# Autodesk Inventor assembly: 05-0010
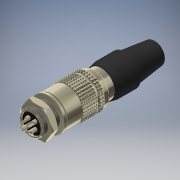
[picture p0: Inventor's stored thumbnail of the model, 180x180]
Saved by Autodesk Inventor 2018 (Build 220112000, 112)
## iProperties
Created: 2019-09-26
Part Number: 05-0010
Document SubType Name: Assembly
Designer: Bradley
Author: Bradley
## Documents named in this file (4)
- C:\Users\Bradley\Documents\GitHub\Resources\SupplierDocuments\05 - Connectors THT\05-0010\05-0010.iam
- C:\Users\Bradley\Documents\GitHub\Resources\SupplierDocuments\05 - Connectors THT\05-0010\05-0010.ipt
- C:\Users\Bradley\Documents\GitHub\Resources\SupplierDocuments\05 - Connectors THT\05-0010P\05-0010P.ipt
- C:\Users\Bradley\Documents\GitHub\Resources\SupplierDocuments\05 - Connectors THT\05-0010\Nut_M8x0.5_2mm.ipt
## Components (3 placed, 3 different names)
1. 05-0010:1 — Mate:2
2. 05-0010P:1
3. Nut_M8x0.5_2mm:1 — Mate:2
## Relationships (4: Mate 2, Insert 1, Flush 1)
- [Insert]: 05-0010:1 ↔ 05-0010P:1
- [Flush]: 05-0010:1 ↔ 05-0010P:1
- [Mate]: 05-0010:1 ↔ Nut_M8x0.5_2mm:1
- Mate:2 (2 mm): 05-0010:1 ↔ Nut_M8x0.5_2mm:1
